# Autodesk Inventor assembly: Ensamble Marcela Meléndez
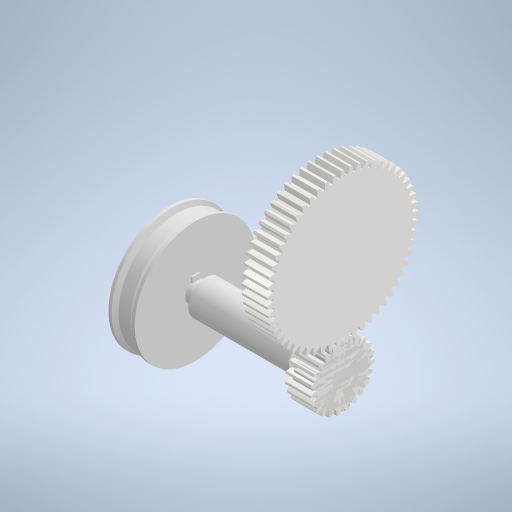
[picture p0: Inventor's stored thumbnail of the model, 512x512]
Saved by Autodesk Inventor 2024 (Build 280153000, 153)
## iProperties
Created: 2024-03-14
Part Number: Ensamble Marcela Meléndez
Document SubType Name: Assembly
Designer: Marcela
Author: Marcela
## Documents named in this file (6)
- C:\Users\Marcela\Documents\TERCER AÑO 2024\QUINTO CICLO 2024\DINÁMICA\DINÁMICA LAB\Ensamble Marcela Meléndez.iam
- C:\Users\Marcela\Documents\TERCER AÑO 2024\QUINTO CICLO 2024\DINÁMICA\POLEA.ipt
- C:\Users\Marcela\Documents\TERCER AÑO 2024\QUINTO CICLO 2024\DINÁMICA\ENGRANE.ipt
- C:\Users\Marcela\Documents\TERCER AÑO 2024\QUINTO CICLO 2024\DINÁMICA\EJE_CUÑEROS.ipt
- C:\Users\Marcela\Documents\TERCER AÑO 2024\QUINTO CICLO 2024\DINÁMICA\CUÑA.ipt
- C:\Users\Marcela\Documents\TERCER AÑO 2024\QUINTO CICLO 2024\DINÁMICA\DINÁMICA LAB\Esamble Marcela Meléndez\Design Accelerator\Spur Gears1.iam
## Components (6 placed, 5 different names)
1. POLEA:1 — Cylindrical:1, Flush:1
2. ENGRANE:1 — Cylindrical:2, Flush:2, Rotational:1
3. EJE_CUÑEROS:1 — Cylindrical:1, Flush:1, Cylindrical:2, Flush:2, Rigid:1, Rigid:2
4. CUÑA:1 — Rigid:1
5. CUÑA:2 — Rigid:2
6. Spur Gears:1 [sub-assembly] — Rotational:1
## Relationships (7: CylindricalJoint 2, Flush 2, WeldJoint 2, RevoluteJoint 1)
- Cylindrical:1: POLEA:1 ↔ EJE_CUÑEROS:1
- Flush:1: POLEA:1 ↔ EJE_CUÑEROS:1
- Cylindrical:2: ENGRANE:1 ↔ EJE_CUÑEROS:1
- Flush:2: ENGRANE:1 ↔ EJE_CUÑEROS:1
- Rigid:1 [WeldJoint]: EJE_CUÑEROS:1 ↔ CUÑA:1
- Rigid:2 [WeldJoint]: EJE_CUÑEROS:1 ↔ CUÑA:2
- Rotational:1 [RevoluteJoint]: ENGRANE:1 ↔ Spur Gears:1
